# Autodesk Inventor assembly: Assembly1
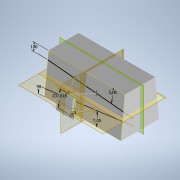
[picture p0: Inventor's stored thumbnail of the model, 180x180]
Saved by Autodesk Inventor 2021 (Build 250183000, 183)
## iProperties
Created: 2021-05-04
Part Number: Assembly1
Document SubType Name: Assembly
Designer: andre
Author: andre
## Documents named in this file (5)
- C:\Users\andre\Desktop\DYNAMIS 2021\Riunioni - Corsi\Corsi Academy\Multibody-Suspension\CAD files\Inventor\Assembly1.iam
- C:\Users\andre\Desktop\DYNAMIS 2021\Riunioni - Corsi\Corsi Academy\Multibody-Suspension\CAD files\Inventor\Telaio.ipt
- C:\Users\andre\Desktop\DYNAMIS 2021\Riunioni - Corsi\Corsi Academy\Multibody-Suspension\CAD files\Inventor\Braccetto.ipt
- C:\Users\andre\Desktop\DYNAMIS 2021\Riunioni - Corsi\Corsi Academy\Multibody-Suspension\CAD files\Inventor\hub.ipt
- C:\Users\andre\Desktop\DYNAMIS 2021\Riunioni - Corsi\Corsi Academy\Multibody-Suspension\CAD files\Inventor\tie.ipt
## Components (5 placed, 4 different names)
1. Telaio:1 — Flush:1, Flush:2, Flush:3, Mate:1, Mate:3
2. Braccetto:1 — Mate:1, Mate:2, Mate:5
3. Braccetto:2 — Mate:3, Mate:4, Mate:6, Mate:8
4. hub:1 — Mate:5, Mate:6, Mate:7, Mate:9
5. tie:1 — Mate:8, Mate:9
## Relationships (12: Mate 9, Flush 3)
- Flush:1: Telaio:1
- Flush:2: Telaio:1
- Flush:3: Telaio:1
- Mate:1: Telaio:1 ↔ Braccetto:1
- Mate:2: Braccetto:1
- Mate:3: Telaio:1 ↔ Braccetto:2
- Mate:4: Braccetto:2
- Mate:5: Braccetto:1 ↔ hub:1
- Mate:6: Braccetto:2 ↔ hub:1
- Mate:7: hub:1
- Mate:8: Braccetto:2 ↔ tie:1
- Mate:9: hub:1 ↔ tie:1
